# Autodesk Inventor assembly: МД.001.100 - База поворотного стола
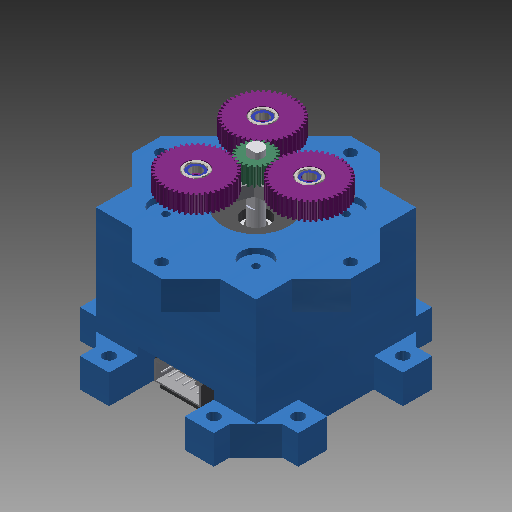
[picture p0: Inventor's stored thumbnail of the model, 512x512]
Saved by Autodesk Inventor 2019 (Build 230136000, 136)
## iProperties
Created: 2019-12-22
Part Number: МД.001.100 - База поворотного стола
Material: Типовые
Document SubType Name: Assembly
Designer: Петров Иван
Author: Петров Иван
## Documents named in this file (6)
- E:\IVAN\Ivan_desktop\GitHub\Arm_manip\hardware\МД.001.100 - База поворотного стола.iam
- E:\IVAN\Ivan_desktop\GitHub\Arm_manip\hardware\МД.001.101 - Стойка мотора.ipt
- E:\IVAN\Ivan_desktop\GitHub\Arm_manip\hardware\Standart_things\Nema 17HS4401-S.ipt
- E:\IVAN\Ivan_desktop\GitHub\Arm_manip\hardware\МД.001.203 - Водило.ipt
- E:\IVAN\Ivan_desktop\GitHub\Arm_manip\hardware\МД.001.204 - Солнечная шестерня.ipt
- E:\IVAN\Ivan_desktop\GitHub\Arm_manip\hardware\МД.001.203_1 - Сателлит с подшипником.iam
## Components (7 placed, 5 different names)
1. МД.001.101 - Стойка мотора:1 — Совмещение:1, Совмещение:2, Совмещение:3
2. Nema 17HS4401-S:1 — Совмещение:1, Совмещение:2, Совмещение:3, Совмещение:14, Совмещение:17
3. МД.001.203 - Водило:1 — Совмещение:14, Совмещение:16, Совмещение:18, Совмещение:19, Совмещение:20, Совмещение:21, Совмещение:22, Совмещение:23
4. МД.001.204 - Солнечная шестерня:1 — Совмещение:16, Совмещение:17
5. МД.001.203_1 - Сателлит с подшипником:1 [sub-assembly] — Совмещение:18, Совмещение:19
6. МД.001.203_1 - Сателлит с подшипником:2 [sub-assembly] — Совмещение:20, Совмещение:21
7. МД.001.203_1 - Сателлит с подшипником:3 [sub-assembly] — Совмещение:22, Совмещение:23
## Relationships (12: Mate 12)
- Совмещение:1 [Mate]: МД.001.101 - Стойка мотора:1 ↔ Nema 17HS4401-S:1
- Совмещение:2 [Mate]: МД.001.101 - Стойка мотора:1 ↔ Nema 17HS4401-S:1
- Совмещение:3 [Mate]: МД.001.101 - Стойка мотора:1 ↔ Nema 17HS4401-S:1
- Совмещение:14 [Mate]: Nema 17HS4401-S:1 ↔ МД.001.203 - Водило:1
- Совмещение:16 [Mate]: МД.001.203 - Водило:1 ↔ МД.001.204 - Солнечная шестерня:1
- Совмещение:17 [Mate]: Nema 17HS4401-S:1 ↔ МД.001.204 - Солнечная шестерня:1
- Совмещение:18 [Mate]: МД.001.203 - Водило:1 ↔ МД.001.203_1 - Сателлит с подшипником:1
- Совмещение:19 [Mate]: МД.001.203 - Водило:1 ↔ МД.001.203_1 - Сателлит с подшипником:1
- Совмещение:20 [Mate]: МД.001.203 - Водило:1 ↔ МД.001.203_1 - Сателлит с подшипником:2
- Совмещение:21 [Mate]: МД.001.203 - Водило:1 ↔ МД.001.203_1 - Сателлит с подшипником:2
- Совмещение:22 [Mate]: МД.001.203 - Водило:1 ↔ МД.001.203_1 - Сателлит с подшипником:3
- Совмещение:23 [Mate]: МД.001.203 - Водило:1 ↔ МД.001.203_1 - Сателлит с подшипником:3
